# Autodesk Inventor assembly: AssemblyV_1
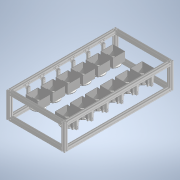
[picture p0: Inventor's stored thumbnail of the model, 180x180]
Saved by Autodesk Inventor 2022 (Build 260153000, 153)
## iProperties
Created: 2022-09-21
Part Number: AssemblyV_1
Document SubType Name: Assembly
Designer: Garrett Raker
Author: Garrett Raker
## Documents named in this file (13)
- F:\College Stuff\ATMAE Robotics\Pill Dispenser Robot\AssemblyV_1.iam
- F:\College Stuff\ATMAE Robotics\Pill Dispenser Robot\Frame Stuff\20x20x600 T Slot Extrusion Bar.ipt
- F:\College Stuff\ATMAE Robotics\Pill Dispenser Robot\Load Cell_Hopper_Connection\Load Cell Hopper Interface.iam
- F:\College Stuff\ATMAE Robotics\Pill Dispenser Robot\Frame Stuff\20x20x600 T Slot Extrusion Bar_MIR.ipt
- F:\College Stuff\ATMAE Robotics\Pill Dispenser Robot\Load Cell_Hopper_Connection\Load Cell Hopper Interface_MIR.iam
- F:\College Stuff\ATMAE Robotics\Pill Dispenser Robot\Frame Stuff\20x20x150 T Slot Extrusion Bar.ipt
- F:\College Stuff\ATMAE Robotics\Pill Dispenser Robot\Frame Stuff\20x20x150 T Slot Extrusion Bar_MIR.ipt
- F:\College Stuff\ATMAE Robotics\Pill Dispenser Robot\Frame Stuff\20x20x600 T Slot Extrusion Bar_MIR1.ipt
- F:\College Stuff\ATMAE Robotics\Pill Dispenser Robot\Frame Stuff\20x20x600 T Slot Extrusion Bar_MIR_MIR.ipt
- F:\College Stuff\ATMAE Robotics\Pill Dispenser Robot\Frame Stuff\20x20x301.4 T Slot Extrusion Bar.ipt
- F:\College Stuff\ATMAE Robotics\Pill Dispenser Robot\Frame Stuff\20x20x301.4 T Slot Extrusion Bar_MIR.ipt
- F:\College Stuff\ATMAE Robotics\Pill Dispenser Robot\Frame Stuff\20x20x301.4 T Slot Extrusion Bar_MIR1.ipt
- F:\College Stuff\ATMAE Robotics\Pill Dispenser Robot\Frame Stuff\20x20x301.4 T Slot Extrusion Bar_MIR_MIR.ipt
## Components (24 placed, 12 different names)
1. 20x20x600 T Slot Extrusion Bar:1 — Mate:1, Mate:2, Mate:6, Flush:3, Flush:4, Flush:7, Mate:9, Flush:8
2. 20x20x600 T Slot Extrusion Bar_MIR:1 — Mate:4, Flush:2, Flush:5, Flush:6, Mate:7, Flush:9, Flush:10, Mate:10
3. 20x20x150 T Slot Extrusion Bar:1 — Mate:6, Flush:3, Flush:4, Flush:14
4. 20x20x150 T Slot Extrusion Bar:2 — Flush:5, Flush:6, Mate:7, Flush:13, Mate:12, Flush:17, Flush:18, Mate:14
5. 20x20x150 T Slot Extrusion Bar_MIR:1 — Flush:7, Mate:9, Flush:8, Flush:11
6. 20x20x150 T Slot Extrusion Bar_MIR:2 — Flush:9, Flush:10, Mate:10, Mate:11, Flush:12, Mate:13, Flush:15, Flush:16
7. 20x20x600 T Slot Extrusion Bar_MIR1:1
8. 20x20x600 T Slot Extrusion Bar_MIR_MIR:1
9. 20x20x301.4 T Slot Extrusion Bar:1 — Mate:11, Flush:11, Flush:12
10. 20x20x301.4 T Slot Extrusion Bar_MIR:1 — Flush:13, Mate:12, Flush:14
11. 20x20x301.4 T Slot Extrusion Bar_MIR1:1 — Mate:13, Flush:15, Flush:16
12. 20x20x301.4 T Slot Extrusion Bar_MIR_MIR:1 — Flush:17, Flush:18, Mate:14
13. Load Cell Hopper Interface:1 [sub-assembly] — Mate:1, Mate:2
14. Load Cell Hopper Interface:2 [sub-assembly]
15. Load Cell Hopper Interface:3 [sub-assembly] — Symmetry:1, Flush:1
16. Load Cell Hopper Interface:4 [sub-assembly] — Symmetry:1
17. Load Cell Hopper Interface:5 [sub-assembly]
18. Load Cell Hopper Interface:6 [sub-assembly]
19. Load Cell Hopper Interface_MIR:1 [sub-assembly] — Mate:4, Flush:2
20. Load Cell Hopper Interface_MIR:2 [sub-assembly]
21. Load Cell Hopper Interface_MIR:3 [sub-assembly] — Symmetry:2, Mate:5
22. Load Cell Hopper Interface_MIR:4 [sub-assembly] — Symmetry:2
23. Load Cell Hopper Interface_MIR:5 [sub-assembly]
24. Load Cell Hopper Interface_MIR:6 [sub-assembly]
## Component patterns: (6 elements, first: Load Cell Hopper Interface:1), (6 elements, first: Load Cell Hopper Interface_MIR:1)
## Relationships (33: Flush 18, Mate 13, Symmetry 2)
- Mate:1: 20x20x600 T Slot Extrusion Bar:1 ↔ Load Cell Hopper Interface:1
- Mate:2: 20x20x600 T Slot Extrusion Bar:1 ↔ Load Cell Hopper Interface:1
- Symmetry:1: Load Cell Hopper Interface:3 ↔ Load Cell Hopper Interface:4
- Mate:3
- Flush:1 (50 mm): Load Cell Hopper Interface:3
- Mate:4: 20x20x600 T Slot Extrusion Bar_MIR:1 ↔ Load Cell Hopper Interface_MIR:1
- Flush:2: 20x20x600 T Slot Extrusion Bar_MIR:1 ↔ Load Cell Hopper Interface_MIR:1
- Symmetry:2: Load Cell Hopper Interface_MIR:3 ↔ Load Cell Hopper Interface_MIR:4
- Mate:5 (50 mm): Load Cell Hopper Interface_MIR:3
- Mate:6: 20x20x600 T Slot Extrusion Bar:1 ↔ 20x20x150 T Slot Extrusion Bar:1
- Flush:3: 20x20x600 T Slot Extrusion Bar:1 ↔ 20x20x150 T Slot Extrusion Bar:1
- Flush:4: 20x20x600 T Slot Extrusion Bar:1 ↔ 20x20x150 T Slot Extrusion Bar:1
- Flush:5: 20x20x600 T Slot Extrusion Bar_MIR:1 ↔ 20x20x150 T Slot Extrusion Bar:2
- Flush:6: 20x20x600 T Slot Extrusion Bar_MIR:1 ↔ 20x20x150 T Slot Extrusion Bar:2
- Mate:7: 20x20x600 T Slot Extrusion Bar_MIR:1 ↔ 20x20x150 T Slot Extrusion Bar:2
- Flush:7: 20x20x600 T Slot Extrusion Bar:1 ↔ 20x20x150 T Slot Extrusion Bar_MIR:1
- Mate:9: 20x20x600 T Slot Extrusion Bar:1 ↔ 20x20x150 T Slot Extrusion Bar_MIR:1
- Flush:8: 20x20x600 T Slot Extrusion Bar:1 ↔ 20x20x150 T Slot Extrusion Bar_MIR:1
- Flush:9: 20x20x600 T Slot Extrusion Bar_MIR:1 ↔ 20x20x150 T Slot Extrusion Bar_MIR:2
- Flush:10: 20x20x600 T Slot Extrusion Bar_MIR:1 ↔ 20x20x150 T Slot Extrusion Bar_MIR:2
- Mate:10: 20x20x600 T Slot Extrusion Bar_MIR:1 ↔ 20x20x150 T Slot Extrusion Bar_MIR:2
- Mate:11: 20x20x150 T Slot Extrusion Bar_MIR:2 ↔ 20x20x301.4 T Slot Extrusion Bar:1
- Flush:11: 20x20x150 T Slot Extrusion Bar_MIR:1 ↔ 20x20x301.4 T Slot Extrusion Bar:1
- Flush:12: 20x20x150 T Slot Extrusion Bar_MIR:2 ↔ 20x20x301.4 T Slot Extrusion Bar:1
- Flush:13: 20x20x150 T Slot Extrusion Bar:2 ↔ 20x20x301.4 T Slot Extrusion Bar_MIR:1
- Mate:12: 20x20x150 T Slot Extrusion Bar:2 ↔ 20x20x301.4 T Slot Extrusion Bar_MIR:1
- Flush:14: 20x20x150 T Slot Extrusion Bar:1 ↔ 20x20x301.4 T Slot Extrusion Bar_MIR:1
- Mate:13: 20x20x150 T Slot Extrusion Bar_MIR:2 ↔ 20x20x301.4 T Slot Extrusion Bar_MIR1:1
- Flush:15: 20x20x150 T Slot Extrusion Bar_MIR:2 ↔ 20x20x301.4 T Slot Extrusion Bar_MIR1:1
- Flush:16: 20x20x150 T Slot Extrusion Bar_MIR:2 ↔ 20x20x301.4 T Slot Extrusion Bar_MIR1:1
- Flush:17: 20x20x150 T Slot Extrusion Bar:2 ↔ 20x20x301.4 T Slot Extrusion Bar_MIR_MIR:1
- Flush:18: 20x20x150 T Slot Extrusion Bar:2 ↔ 20x20x301.4 T Slot Extrusion Bar_MIR_MIR:1
- Mate:14: 20x20x150 T Slot Extrusion Bar:2 ↔ 20x20x301.4 T Slot Extrusion Bar_MIR_MIR:1
